# Autodesk Inventor assembly: MC15A_V5
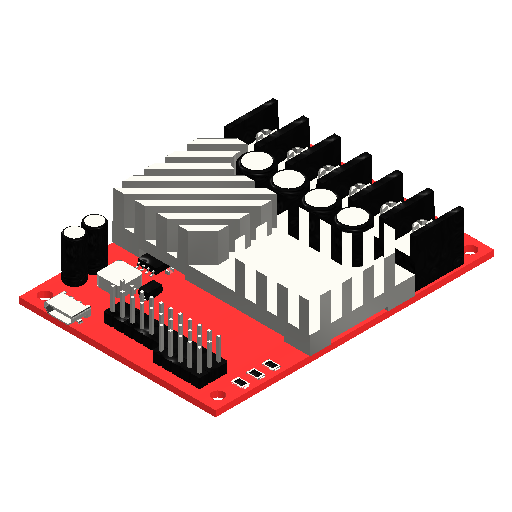
[picture p0: Inventor's stored thumbnail of the model, 512x512]
Saved by Autodesk Inventor 2026.1 (Build 301233000, 233)
## iProperties
Created: 2015-07-01
Part Number: MC15A_V5
Description: SolidWorks IGES file using analytic representation for surfaces
Document SubType Name: Assembly
Designer: gianm
Sending System: SolidWorks 2013
Preprocessor: SolidWorks 2013
Minimum Resolution: 0.0
Sending System Product ID: MC15A-V5
Receiving System Product ID: MC15A-V5
Sent Units: Millimeter
Translation Standard: IGES 5.3
Model Creation Time: 2015-07-01
Title: C:\Users\A Vinh\Desktop\MC15A-V5.IGS
Author: A Vinh
## Documents named in this file (18)
- D:\Tesis\Modelo 3D\CAD\Electronicos\MC15A_V5\MC15A_V5\MC15A_V5\MC15A_V5.iam
- D:\Tesis\Modelo 3D\CAD\Electronicos\MC15A_V5\MC15A_V5\MC15A_V5\MCV30A-PCB.ipt
- D:\Tesis\Modelo 3D\CAD\Electronicos\MC15A_V5\MC15A_V5\MC15A_V5\ED2949-ND.ipt
- D:\Tesis\Modelo 3D\CAD\Electronicos\MC15A_V5\MC15A_V5\MC15A_V5\P15369TB-ND.ipt
- D:\Tesis\Modelo 3D\CAD\Electronicos\MC15A_V5\MC15A_V5\MC15A_V5\LM22676MRE-5.0_NOPBTR-ND.ipt
- D:\Tesis\Modelo 3D\CAD\Electronicos\MC15A_V5\MC15A_V5\MC15A_V5\SSA34-E3_61TGICT-ND.ipt
- D:\Tesis\Modelo 3D\CAD\Electronicos\MC15A_V5\MC15A_V5\MC15A_V5\609-4618-1-ND.ipt
- D:\Tesis\Modelo 3D\CAD\Electronicos\MC15A_V5\MC15A_V5\MC15A_V5\P16851CT-ND.ipt
- D:\Tesis\Modelo 3D\CAD\Electronicos\MC15A_V5\MC15A_V5\MC15A_V5\SRP7030-8R2FMCT-ND.ipt
- D:\Tesis\Modelo 3D\CAD\Electronicos\MC15A_V5\MC15A_V5\MC15A_V5\P833-ND.ipt
- D:\Tesis\Modelo 3D\CAD\Electronicos\MC15A_V5\MC15A_V5\MC15A_V5\PBC09DAAN.ipt
- D:\Tesis\Modelo 3D\CAD\Electronicos\MC15A_V5\MC15A_V5\MC15A_V5\PBC02DAAN.ipt
- D:\Tesis\Modelo 3D\CAD\Electronicos\MC15A_V5\MC15A_V5\MC15A_V5\PBC05SAAN.ipt
- D:\Tesis\Modelo 3D\CAD\Electronicos\MC15A_V5\MC15A_V5\MC15A_V5\CRF2512-FV-R001ELFCT-ND.ipt
- D:\Tesis\Modelo 3D\CAD\Electronicos\MC15A_V5\MC15A_V5\MC15A_V5\620-1319-1-ND.ipt
- D:\Tesis\Modelo 3D\CAD\Electronicos\MC15A_V5\MC15A_V5\MC15A_V5\ATXMEGA32A4U-AU-ND.ipt
- D:\Tesis\Modelo 3D\CAD\Electronicos\MC15A_V5\MC15A_V5\MC15A_V5\MC30A_HeatSink_V5.ipt
- D:\Tesis\Modelo 3D\CAD\Electronicos\MC15A_V5\MC15A_V5\MC15A_V5\311-1366-2-ND.ipt
## Components (25 placed, 17 different names)
1. MCV30A-PCB
2. ED2949-ND
3. P15369TB-ND
4. LM22676MRE-5.0_NOPBTR-ND
5. SSA34-E3_61TGICT-ND
6. 609-4618-1-ND
7. P16851CT-ND
8. P16851CT-ND:1
9. P16851CT-ND:2
10. SRP7030-8R2FMCT-ND
11. P833-ND
12. P833-ND:1
13. PBC09DAAN
14. PBC02DAAN
15. PBC05SAAN
16. CRF2512-FV-R001ELFCT-ND
17. CRF2512-FV-R001ELFCT-ND:1
18. 620-1319-1-ND
19. 620-1319-1-ND:1
20. ATXMEGA32A4U-AU-ND
21. MC30A_HeatSink_V5
22. P15369TB-ND:1
23. P15369TB-ND:2
24. P15369TB-ND:3
25. 311-1366-2-ND
## Named parameters: Finish1_Area = 80.6299, Finish2_Area = 101.827, Finish3_Area = 54.0108
note: some values were not read from the file. Shown as the stored number, unit unknown: "Finish1_Area", "Finish2_Area", "Finish3_Area".
